# Autodesk Inventor assembly: Widelec
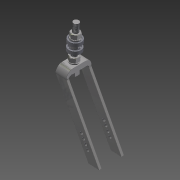
[picture p0: Inventor's stored thumbnail of the model, 180x180]
Saved by Autodesk Inventor 2015 (Build 190159000, 159)
## iProperties
Created: 2016-01-12
Part Number: Widelec
Document SubType Name: Assembly
Designer: graaapsik
Author: graaapsik
## Documents named in this file (7)
- C:\Users\EriveltonDell\Documents\Centro Universitário da FEI\Wheelchair\CADEIRA DE RODAS - DESENHO\Model\Widelec.iam
- C:\Users\EriveltonDell\Documents\Centro Universitário da FEI\Wheelchair\CADEIRA DE RODAS - DESENHO\Model\Widelec.ipt
- C:\Users\EriveltonDell\Documents\Centro Universitário da FEI\Wheelchair\CADEIRA DE RODAS - DESENHO\Model\Śruba_do_widelca.ipt
- C:\Users\EriveltonDell\Documents\Centro Universitário da FEI\Wheelchair\CADEIRA DE RODAS - DESENHO\Model\ISO 7092 - ST 12 - 140 HV.ipt
- C:\Users\EriveltonDell\Documents\Centro Universitário da FEI\Wheelchair\CADEIRA DE RODAS - DESENHO\Model\ISO 4032 - M12ISO.ipt
- C:\Users\EriveltonDell\Documents\Centro Universitário da FEI\Wheelchair\CADEIRA DE RODAS - DESENHO\Model\Rolling bearing QJ1001 GB_T 294-94.ipt
- C:\Users\EriveltonDell\Documents\Centro Universitário da FEI\Wheelchair\CADEIRA DE RODAS - DESENHO\Model\Separator_do_widelca.ipt
## Components (12 placed, 6 different names)
1. Śruba_do_widelca:1 — Zestawiający:3, Zestawiający:5, Zestawiający:6, Zestawiający:11, Zestawiający:13, Zestawiający:15, Zestawiający:17, Zestawiający:21
2. Widelec:1 — Zestawiający:4, Zestawiający:5, Zestawiający:7
3. ISO 7092 ST 12 - 140 HV:1 — Zestawiający:16, Zestawiający:17
4. ISO 7092 ST 12 - 140 HV:2 — Zestawiający:3, Zestawiający:4, Wstaw:1
5. ISO 7092 ST 12 - 140 HV:3 — Zestawiający:11, Zestawiający:14, Wstaw:3
6. ISO 7092 ST 12 - 140 HV:4 — Zestawiający:6, Zestawiający:7, Wstaw:2
7. Rolling bearing GB/T 294-1994 QJ1001:1 — Zestawiający:15, Zestawiający:16
8. Rolling bearing GB/T 294-1994 QJ1001:2 — Zestawiający:13, Zestawiający:14, Zestawiający:20
9. Separator_do_widelca:1 — Zestawiający:20, Zestawiający:21
10. ISO 4032 M12:4 — Wstaw:1
11. ISO 4032 M12:5 — Wstaw:2
12. ISO 4032 M12:6 — Wstaw:3
## Relationships (16: Mate 13, Insert 3)
- Zestawiający:3 [Mate]: Śruba_do_widelca:1 ↔ ISO 7092 ST 12 - 140 HV:2
- Zestawiający:4 [Mate]: Widelec:1 ↔ ISO 7092 ST 12 - 140 HV:2
- Zestawiający:5 [Mate]: Śruba_do_widelca:1 ↔ Widelec:1
- Zestawiający:6 [Mate]: Śruba_do_widelca:1 ↔ ISO 7092 ST 12 - 140 HV:4
- Zestawiający:7 [Mate]: Widelec:1 ↔ ISO 7092 ST 12 - 140 HV:4
- Zestawiający:11 [Mate]: Śruba_do_widelca:1 ↔ ISO 7092 ST 12 - 140 HV:3
- Zestawiający:13 [Mate]: Śruba_do_widelca:1 ↔ Rolling bearing GB/T 294-1994 QJ1001:2
- Zestawiający:14 [Mate]: ISO 7092 ST 12 - 140 HV:3 ↔ Rolling bearing GB/T 294-1994 QJ1001:2
- Zestawiający:15 [Mate]: Śruba_do_widelca:1 ↔ Rolling bearing GB/T 294-1994 QJ1001:1
- Zestawiający:16 [Mate]: ISO 7092 ST 12 - 140 HV:1 ↔ Rolling bearing GB/T 294-1994 QJ1001:1
- Zestawiający:17 [Mate]: Śruba_do_widelca:1 ↔ ISO 7092 ST 12 - 140 HV:1
- Zestawiający:20 [Mate]: Rolling bearing GB/T 294-1994 QJ1001:2 ↔ Separator_do_widelca:1
- Zestawiający:21 [Mate]: Śruba_do_widelca:1 ↔ Separator_do_widelca:1
- Wstaw:1 [Insert]: ISO 7092 ST 12 - 140 HV:2 ↔ ISO 4032 M12:4
- Wstaw:2 [Insert]: ISO 7092 ST 12 - 140 HV:4 ↔ ISO 4032 M12:5
- Wstaw:3 [Insert]: ISO 7092 ST 12 - 140 HV:3 ↔ ISO 4032 M12:6
